# Autodesk Inventor assembly: 2021-2022 Grabber Module
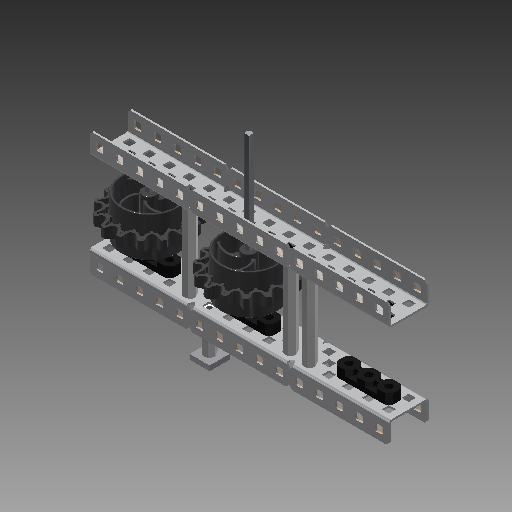
[picture p0: Inventor's stored thumbnail of the model, 512x512]
Saved by Autodesk Inventor 2019 (Build 230136000, 136)
## iProperties
Created: 2021-09-17
Part Number: 2021-2022 Grabber Module
Document SubType Name: Assembly
Designer: 22spencen
Author: 22spencen
## Documents named in this file (9)
- \\Chopper\2022\22spencen\Documents\VEX_CAD\Assemblies\2021-2022 Grabber Module.iam
- \\Chopper\2022\22spencen\Documents\VEX_CAD\Part Files\VEX Parts Library 2016\Imperial\Structure\C-Channel 1x2x1x15 Hole.ipt
- \\Chopper\2022\22spencen\Documents\VEX_CAD\Part Files\VEX Parts Library 2016\Imperial\Motion\Bearing Flat.ipt
- \\Chopper\2022\22spencen\Documents\VEX_CAD\Part Files\VEX Parts Library 2016\Imperial\Structure\2 inch Standoff.ipt
- \\Chopper\2022\22spencen\Documents\VEX_CAD\Part Files\VEX Parts Library 2016\Imperial\Motion\Shaft 2 inch.ipt
- \\Chopper\2022\22spencen\Documents\VEX_CAD\Part Files\VEX Parts Library 2016\Imperial\Motion\Shaft 4 inch.ipt
- \\Chopper\2022\22spencen\Documents\VEX_CAD\Part Files\VEX Parts Library 2016\Imperial\Motion\Sprockets and Chain\Tank Tread Drive Wheel.ipt
- \\Chopper\2022\22spencen\Documents\VEX_CAD\Part Files\VEX Parts Library 2016\Imperial\Structure\1 inch Standoff.ipt
- \\Chopper\2022\22spencen\Documents\VEX_CAD\Assemblies\PlaceholderPart.ipt
## Components (17 placed, 8 different names)
1. C-Channel 1x2x1x15 Hole:1 — Mate:1, Mate:2, Mate:3, Tangent:1, Mate:4, Tangent:2, Mate:5, Tangent:3, Mate:6, Flush:1, Flush:2, Mate:15
2. Bearing Flat:1 — Mate:1, Flush:7, Flush:8
3. Bearing Flat:2 — Mate:2, Insert:2
4. Bearing Flat:3 — Mate:3, Flush:3, Flush:4
5. 2 inch Standoff:1 — Tangent:1, Mate:4
6. 2 inch Standoff:2 — Tangent:2, Mate:5, Mate:7
7. 2 inch Standoff:3 — Tangent:3, Mate:6
8. C-Channel 1x2x1x15 Hole:2 — Flush:1, Flush:2, Mate:7, Mate:8, Mate:9, Mate:10
9. Bearing Flat:4 — Flush:3, Flush:4, Mate:8
10. Bearing Flat:5 — Flush:7, Flush:8, Mate:10, Insert:1
11. Bearing Flat:6 — Mate:9
12. Shaft 2 inch:1 — Insert:1, Mate:11, Mate:12
13. Shaft 4 inch:1 — Insert:2, Mate:13, Mate:14
14. Tank Tread Drive Wheel:1 — Mate:11, Mate:12, Flush:9
15. Tank Tread Drive Wheel:2 — Mate:13, Mate:14, Flush:9
16. 1 inch Standoff:1 — Mate:15, Flush:10
17. PlaceholderPart:1 — Flush:10
## Relationships (28: Mate 15, Flush 8, Tangent 3, Insert 2)
- Mate:1: C-Channel 1x2x1x15 Hole:1 ↔ Bearing Flat:1
- Mate:2: C-Channel 1x2x1x15 Hole:1 ↔ Bearing Flat:2
- Mate:3: C-Channel 1x2x1x15 Hole:1 ↔ Bearing Flat:3
- Tangent:1: C-Channel 1x2x1x15 Hole:1 ↔ 2 inch Standoff:1
- Mate:4: C-Channel 1x2x1x15 Hole:1 ↔ 2 inch Standoff:1
- Tangent:2: C-Channel 1x2x1x15 Hole:1 ↔ 2 inch Standoff:2
- Mate:5: C-Channel 1x2x1x15 Hole:1 ↔ 2 inch Standoff:2
- Tangent:3: C-Channel 1x2x1x15 Hole:1 ↔ 2 inch Standoff:3
- Mate:6: C-Channel 1x2x1x15 Hole:1 ↔ 2 inch Standoff:3
- Flush:1: C-Channel 1x2x1x15 Hole:1 ↔ C-Channel 1x2x1x15 Hole:2
- Flush:2: C-Channel 1x2x1x15 Hole:1 ↔ C-Channel 1x2x1x15 Hole:2
- Mate:7: 2 inch Standoff:2 ↔ C-Channel 1x2x1x15 Hole:2
- Flush:3: Bearing Flat:3 ↔ Bearing Flat:4
- Flush:4: Bearing Flat:3 ↔ Bearing Flat:4
- Mate:8: C-Channel 1x2x1x15 Hole:2 ↔ Bearing Flat:4
- Mate:9: C-Channel 1x2x1x15 Hole:2 ↔ Bearing Flat:6
- Flush:7: Bearing Flat:1 ↔ Bearing Flat:5
- Flush:8: Bearing Flat:1 ↔ Bearing Flat:5
- Mate:10: C-Channel 1x2x1x15 Hole:2 ↔ Bearing Flat:5
- Insert:1 (-6.35 mm): Bearing Flat:5 ↔ Shaft 2 inch:1
- Insert:2 (-6.35 mm): Bearing Flat:2 ↔ Shaft 4 inch:1
- Mate:11: Shaft 2 inch:1 ↔ Tank Tread Drive Wheel:1
- Mate:12: Shaft 2 inch:1 ↔ Tank Tread Drive Wheel:1
- Mate:13: Shaft 4 inch:1 ↔ Tank Tread Drive Wheel:2
- Mate:14: Shaft 4 inch:1 ↔ Tank Tread Drive Wheel:2
- Flush:9: Tank Tread Drive Wheel:1 ↔ Tank Tread Drive Wheel:2
- Mate:15: C-Channel 1x2x1x15 Hole:1 ↔ 1 inch Standoff:1
- Flush:10: 1 inch Standoff:1 ↔ PlaceholderPart:1
